# Autodesk Inventor assembly: TestBench_Top.ipt
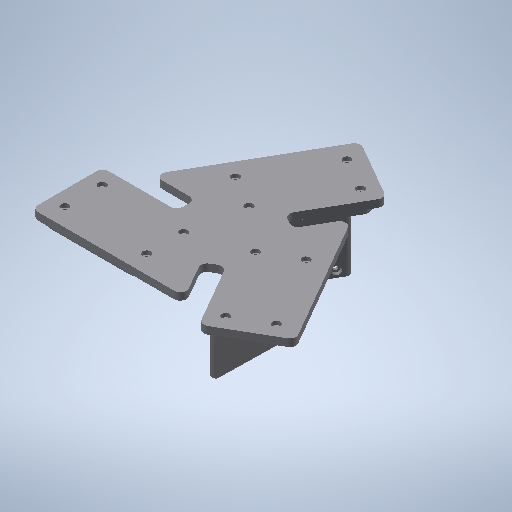
[picture p0: Inventor's stored thumbnail of the model, 512x512]
Saved by Autodesk Inventor 2025.4 (Build 294407000, 407)
## iProperties
Created: 2026-05-15
Part Number: TestBench_Top.ipt
Document SubType Name: Assembly
Designer: louis
Author: louis
## Documents named in this file (3)
- C:\Users\louis\OneDrive\Desktop\R_Trident\02_CAD\07_Test_Bench\TestBench_Top.ipt.iam
- C:\Users\louis\OneDrive\Desktop\R_Trident\02_CAD\07_Test_Bench\TestBench_Top_Motor_Support.ipt
- C:\Users\louis\OneDrive\Desktop\R_Trident\02_CAD\07_Test_Bench\Nema17Mount.ipt
## Components (4 placed, 2 different names)
1. TestBench_Top_Motor_Support:1 — Mate:1, Mate:2, Mate:3, Mate:4, Mate:5, Mate:6, Mate:7, Mate:8, Mate:9
2. Nema17Mount:1 — Mate:1, Mate:2
3. Nema17Mount:2 — Mate:3, Mate:4
4. Nema17Mount:3 — Mate:5, Mate:6
## Relationships (9: Mate 9)
- Mate:1: TestBench_Top_Motor_Support:1 ↔ Nema17Mount:1
- Mate:2: TestBench_Top_Motor_Support:1 ↔ Nema17Mount:1
- Mate:3: TestBench_Top_Motor_Support:1 ↔ Nema17Mount:2
- Mate:4: TestBench_Top_Motor_Support:1 ↔ Nema17Mount:2
- Mate:5: TestBench_Top_Motor_Support:1 ↔ Nema17Mount:3
- Mate:6: TestBench_Top_Motor_Support:1 ↔ Nema17Mount:3
- Mate:7: TestBench_Top_Motor_Support:1
- Mate:8: TestBench_Top_Motor_Support:1
- Mate:9: TestBench_Top_Motor_Support:1
